# Autodesk Inventor assembly: s-assy-unit-bearing
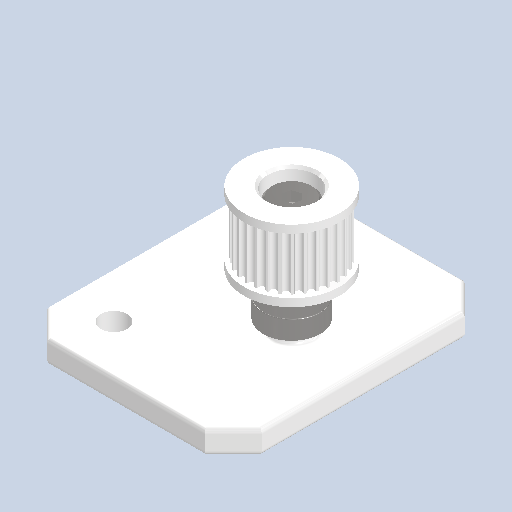
[picture p0: Inventor's stored thumbnail of the model, 512x512]
Saved by Autodesk Inventor 2022 (Build 260153000, 153)
## iProperties
Created: 2022-06-14
Part Number: s-assy-unit-bearing
Document SubType Name: Assembly
Designer: yuto6
Author: yuto6
## Documents named in this file (3)
- C:\Users\yuto6\Documents\CAD\book-reader\s-assy-unit-bearing.iam
- C:\Users\yuto6\Documents\CAD\book-reader\base3.ipt
- C:\Users\yuto6\Documents\CAD\book-reader\s-assy-idler1.iam
## Components (2 placed, 2 different names)
1. base3:1 — メイト:1, メイト:2
2. s-assy-idler1:1 [sub-assembly] — メイト:1, メイト:2
## Relationships (2: Mate 2)
- メイト:1 [Mate]: base3:1 ↔ s-assy-idler1:1
- メイト:2 [Mate]: base3:1 ↔ s-assy-idler1:1
